# Autodesk Inventor assembly: Suporte Inferior
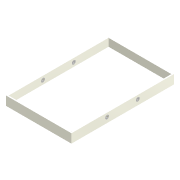
[picture p0: Inventor's stored thumbnail of the model, 180x180]
Saved by Autodesk Inventor 2020 (Build 240168000, 168)
## iProperties
Created: 2021-09-22
Part Number: Suporte Inferior
Document SubType Name: Assembly
Designer: pablo
Author: pablo
## Documents named in this file (5)
- C:\Google Drive\Pablo Arquivos\Projetos\Utilidades Domesticas\Talheres\Suporte Inferior.iam
- C:\Google Drive\Pablo Arquivos\Projetos\Utilidades Domesticas\Talheres\base inferior.ipt
- C:\Google Drive\Pablo Arquivos\Projetos\Utilidades Domesticas\Talheres\Divisória-30cm c rolamento - inferior.ipt
- C:\Google Drive\Pablo Arquivos\Projetos\Utilidades Domesticas\Talheres\Third\AIS2019\SKF_619_6-2Z.iam
- C:\Google Drive\Pablo Arquivos\Projetos\Utilidades Domesticas\Talheres\Divisória-25cm.ipt
## Components (9 placed, 4 different names)
1. base inferior:1 — Mate:13, Mate:14, Mate:15, Mate:16, Mate:17, Mate:18, Mate:19, Mate:20, Mate:23, Mate:24
2. Divisória-30cm c rolamento - inferior:1 — Mate:19, Mate:20, Mate:21, Mate:22
3. Divisória-30cm c rolamento - inferior:2 — Mate:23, Mate:24, Mate:25, Mate:26
4. SKF_619_6-2Z:1 [sub-assembly] — Mate:22
5. SKF_619_6-2Z:2 [sub-assembly] — Mate:21
6. SKF_619_6-2Z:3 [sub-assembly] — Mate:26
7. SKF_619_6-2Z:4 [sub-assembly] — Mate:25
8. Divisória-25cm:1 — Mate:13, Mate:14, Mate:17, Mate:18
9. Divisória-25cm:2 — Mate:15, Mate:16
## Relationships (14: Mate 14)
- Mate:13: base inferior:1 ↔ Divisória-25cm:1
- Mate:14: base inferior:1 ↔ Divisória-25cm:1
- Mate:15: base inferior:1 ↔ Divisória-25cm:2
- Mate:16: base inferior:1 ↔ Divisória-25cm:2
- Mate:17: base inferior:1 ↔ Divisória-25cm:1
- Mate:18: base inferior:1 ↔ Divisória-25cm:1
- Mate:19: base inferior:1 ↔ Divisória-30cm c rolamento - inferior:1
- Mate:20: base inferior:1 ↔ Divisória-30cm c rolamento - inferior:1
- Mate:21: Divisória-30cm c rolamento - inferior:1 ↔ SKF_619_6-2Z:2
- Mate:22: Divisória-30cm c rolamento - inferior:1 ↔ SKF_619_6-2Z:1
- Mate:23: base inferior:1 ↔ Divisória-30cm c rolamento - inferior:2
- Mate:24: base inferior:1 ↔ Divisória-30cm c rolamento - inferior:2
- Mate:25: Divisória-30cm c rolamento - inferior:2 ↔ SKF_619_6-2Z:4
- Mate:26: Divisória-30cm c rolamento - inferior:2 ↔ SKF_619_6-2Z:3
